# Autodesk Inventor assembly: Gantry1
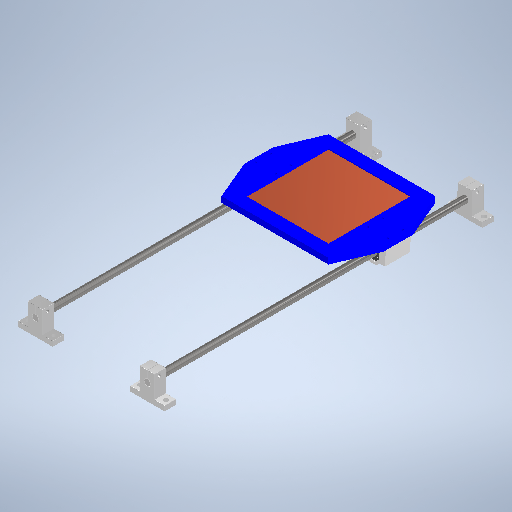
[picture p0: Inventor's stored thumbnail of the model, 512x512]
Saved by Autodesk Inventor 2025.2 (Build 292293000, 293)
## iProperties
Created: 2025-05-31
Part Number: Gantry1
Document SubType Name: Assembly
Designer: Simon
Author: Simon
## Documents named in this file (7)
- C:\Users\Simon\Projects\Hydrogel-3D-Printer\Hardware\Bioprinter Machine Design\Gantry Concept 1\Gantry1.iam
- C:\Users\Simon\Projects\Hydrogel-3D-Printer\Hardware\Bioprinter Machine Design\Gantry Concept 1\SteelShaft_400mm.ipt
- C:\Users\Simon\Projects\Hydrogel-3D-Printer\Hardware\Bioprinter Machine Design\PartsFolder\SK8_LinearShaftSupport.ipt
- C:\Users\Simon\Projects\Hydrogel-3D-Printer\Hardware\Bioprinter Machine Design\PartsFolder\PeltierTEC1_12706.ipt
- C:\Users\Simon\Projects\Hydrogel-3D-Printer\Hardware\Bioprinter Machine Design\PartsFolder\SC8UU\SC8UU.iam
- C:\Users\Simon\Projects\Hydrogel-3D-Printer\Hardware\Bioprinter Machine Design\Gantry Concept 1\BedPlate.ipt
- C:\Users\Simon\Projects\Hydrogel-3D-Printer\Hardware\Bioprinter Machine Design\Gantry Concept 1\BedHousingFrame.ipt
## Components (11 placed, 6 different names)
1. SteelShaft_400mm:1 — Mate:1, Mate:3, Flush:1, Flush:4, Mate:5
2. SteelShaft_400mm:2 — Mate:2, Mate:4, Flush:2, Flush:3, Mate:6
3. SK8_LinearShaftSupport:1 — Mate:1, Flush:1, Flush:5, Flush:6
4. SK8_LinearShaftSupport:2 — Mate:2, Flush:2, Flush:5, Flush:6, Mate:15
5. SK8_LinearShaftSupport:3 — Mate:3, Flush:4, Mate:13, Mate:16
6. SK8_LinearShaftSupport:4 — Mate:4, Flush:3, Mate:14
7. PeltierTEC1_12706:1 — Mate:7, Flush:7, Flush:8
8. SC8UU:1 [sub-assembly] — Mate:5, Mate:11, Flush:9, Flush:11, Flush:12
9. SC8UU:2 [sub-assembly] — Mate:6, Flush:10, Mate:12, Flush:11
10. BedPlate:1 — Mate:7, Flush:7, Flush:8, Mate:8, Mate:9, Mate:10
11. BedHousingFrame:1 — Mate:8, Mate:9, Mate:10, Mate:11, Flush:9, Flush:10, Mate:12, Flush:12
## Relationships (28: Mate 16, Flush 12)
- Mate:1: SteelShaft_400mm:1 ↔ SK8_LinearShaftSupport:1
- Mate:2: SteelShaft_400mm:2 ↔ SK8_LinearShaftSupport:2
- Mate:3: SteelShaft_400mm:1 ↔ SK8_LinearShaftSupport:3
- Mate:4: SteelShaft_400mm:2 ↔ SK8_LinearShaftSupport:4
- Flush:1: SteelShaft_400mm:1 ↔ SK8_LinearShaftSupport:1
- Flush:2: SteelShaft_400mm:2 ↔ SK8_LinearShaftSupport:2
- Flush:3: SteelShaft_400mm:2 ↔ SK8_LinearShaftSupport:4
- Flush:4: SteelShaft_400mm:1 ↔ SK8_LinearShaftSupport:3
- Flush:5: SK8_LinearShaftSupport:1 ↔ SK8_LinearShaftSupport:2
- Flush:6: SK8_LinearShaftSupport:1 ↔ SK8_LinearShaftSupport:2
- Mate:5: SteelShaft_400mm:1 ↔ SC8UU:1
- Mate:6: SteelShaft_400mm:2 ↔ SC8UU:2
- Mate:7: PeltierTEC1_12706:1 ↔ BedPlate:1
- Flush:7 (-30 mm): PeltierTEC1_12706:1 ↔ BedPlate:1
- Flush:8 (30 mm): PeltierTEC1_12706:1 ↔ BedPlate:1
- Mate:8: BedPlate:1 ↔ BedHousingFrame:1
- Mate:9: BedPlate:1 ↔ BedHousingFrame:1
- Mate:10: BedPlate:1 ↔ BedHousingFrame:1
- Mate:11: SC8UU:1 ↔ BedHousingFrame:1
- Flush:9: SC8UU:1 ↔ BedHousingFrame:1
- Flush:10: SC8UU:2 ↔ BedHousingFrame:1
- Mate:12: SC8UU:2 ↔ BedHousingFrame:1
- Mate:13: SK8_LinearShaftSupport:3
- Mate:14: SK8_LinearShaftSupport:4
- Mate:15: SK8_LinearShaftSupport:2
- Mate:16: SK8_LinearShaftSupport:3
- Flush:11: SC8UU:1 ↔ SC8UU:2
- Flush:12 (50 mm): SC8UU:1 ↔ BedHousingFrame:1
